# Autodesk Inventor assembly: FullField-ver2-1111-2021
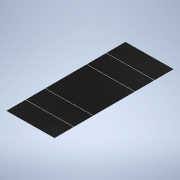
[picture p0: Inventor's stored thumbnail of the model, 180x180]
Saved by Autodesk Inventor 2021 (Build 250183000, 183)
## iProperties
Created: 2021-02-23
Part Number: FullField-ver2-1111-2021
Document SubType Name: Assembly
Designer: CMurray
Author: CMurray
## Documents named in this file (5)
- F:\PHRC CADD 2021\2021 Game Design Challenge\Full Field\Final Assembly\FullField-ver2-1111-2021.iam
- F:\PHRC CADD 2021\2021 Game Design Challenge\Full Field\Parts\FieldFloor-ver1-1111-2021.ipt
- F:\PHRC CADD 2021\2021 Game Design Challenge\Full Field\Parts\Tape\Tape.ipt
- F:\PHRC CADD 2021\2021 Game Design Challenge\Full Field\Parts\Tape\RedAllianceTape-ver1-1111-2021.ipt
- F:\PHRC CADD 2021\2021 Game Design Challenge\Full Field\Parts\Tape\BlueAllianceTape-ver1-1111-2021.ipt
## Components (10 placed, 4 different names)
1. FieldFloor-ver1-1111-2021:1 — Flush:1, Flush:2, Mate:1, Mate:3, Mate:10, Flush:10, Mate:14, Flush:12
2. FieldFloor-ver1-1111-2021:2 — Flush:1, Flush:2, Mate:1, Mate:2, Flush:3, Flush:4, Flush:5, Flush:6, Mate:4, Flush:7, Mate:6, Flush:8, Mate:8, Flush:9, Mate:12, Flush:11
3. Tape:1 — Mate:2, Flush:3, Flush:4, Mate:5, Mate:9, Mate:11
4. Tape:2 — Mate:3, Flush:5, Flush:6, Mate:7, Mate:13, Mate:15
5. Tape:3 — Mate:4, Flush:7, Mate:5
6. Tape:4 — Mate:6, Flush:8, Mate:7
7. RedAllianceTape-ver1-1111-2021:1 — Mate:8, Flush:9, Mate:9
8. RedAllianceTape-ver1-1111-2021:2 — Mate:10, Flush:10, Mate:11
9. BlueAllianceTape-ver1-1111-2021:1 — Mate:12, Flush:11, Mate:13
10. BlueAllianceTape-ver1-1111-2021:2 — Mate:14, Flush:12, Mate:15
## Relationships (27: Mate 15, Flush 12)
- Flush:1: FieldFloor-ver1-1111-2021:1 ↔ FieldFloor-ver1-1111-2021:2
- Flush:2: FieldFloor-ver1-1111-2021:1 ↔ FieldFloor-ver1-1111-2021:2
- Mate:1: FieldFloor-ver1-1111-2021:1 ↔ FieldFloor-ver1-1111-2021:2
- Mate:2: FieldFloor-ver1-1111-2021:2 ↔ Tape:1
- Flush:3: FieldFloor-ver1-1111-2021:2 ↔ Tape:1
- Flush:4 (3606.8 mm): FieldFloor-ver1-1111-2021:2 ↔ Tape:1
- Mate:3: FieldFloor-ver1-1111-2021:1 ↔ Tape:2
- Flush:5: FieldFloor-ver1-1111-2021:2 ↔ Tape:2
- Flush:6 (3606.8 mm): FieldFloor-ver1-1111-2021:2 ↔ Tape:2
- Mate:4: FieldFloor-ver1-1111-2021:2 ↔ Tape:3
- Flush:7: FieldFloor-ver1-1111-2021:2 ↔ Tape:3
- Mate:5 (3657.6 mm): Tape:1 ↔ Tape:3
- Mate:6: FieldFloor-ver1-1111-2021:2 ↔ Tape:4
- Flush:8: FieldFloor-ver1-1111-2021:2 ↔ Tape:4
- Mate:7 (3657.6 mm): Tape:2 ↔ Tape:4
- Mate:8: FieldFloor-ver1-1111-2021:2 ↔ RedAllianceTape-ver1-1111-2021:1
- Flush:9: FieldFloor-ver1-1111-2021:2 ↔ RedAllianceTape-ver1-1111-2021:1
- Mate:9: Tape:1 ↔ RedAllianceTape-ver1-1111-2021:1
- Mate:10: FieldFloor-ver1-1111-2021:1 ↔ RedAllianceTape-ver1-1111-2021:2
- Flush:10: FieldFloor-ver1-1111-2021:1 ↔ RedAllianceTape-ver1-1111-2021:2
- Mate:11: Tape:1 ↔ RedAllianceTape-ver1-1111-2021:2
- Mate:12: FieldFloor-ver1-1111-2021:2 ↔ BlueAllianceTape-ver1-1111-2021:1
- Flush:11: FieldFloor-ver1-1111-2021:2 ↔ BlueAllianceTape-ver1-1111-2021:1
- Mate:13: Tape:2 ↔ BlueAllianceTape-ver1-1111-2021:1
- Mate:14: FieldFloor-ver1-1111-2021:1 ↔ BlueAllianceTape-ver1-1111-2021:2
- Flush:12: FieldFloor-ver1-1111-2021:1 ↔ BlueAllianceTape-ver1-1111-2021:2
- Mate:15: Tape:2 ↔ BlueAllianceTape-ver1-1111-2021:2
